# Autodesk Inventor assembly: Mechanizm
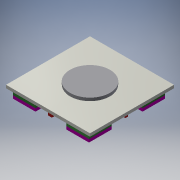
[picture p0: Inventor's stored thumbnail of the model, 180x180]
Saved by Autodesk Inventor 2018 (Build 220112000, 112)
## iProperties
Created: 2018-10-22
Part Number: Mechanizm
Material: Ogólny
Document SubType Name: Assembly
Designer: EWA
Author: EWA
## Documents named in this file (7)
- C:\Users\EWA\Documents\Inventor\Kostka\Mechanizm.iam
- C:\Users\EWA\Documents\Inventor\Kostka\Zamek_II_klucz.ipt
- C:\Users\EWA\Documents\Inventor\Kostka\Pokrywka.ipt
- C:\Users\EWA\Documents\Inventor\Kostka\zamek_II_boki.ipt
- C:\Users\EWA\Documents\Inventor\Kostka\Zamek_I.ipt
- C:\Users\EWA\Documents\Inventor\Kostka\Sciana_pokrywka_168x168.ipt
- C:\Users\EWA\Documents\Inventor\Kostka\Uchwyt_80.ipt
## Components (9 placed, 6 different names)
1. Pokrywka:1 — Zestawiający:1, Równoległy:1, Równoległy:2, Obrotowe:1, Zestawiający:2, Zestawiający:3, Równoległy:3, Równoległy:4, Równoległy:5, Równoległy:6, Zestawiający:4, Zestawiający:5, Równoległy:7, Równoległy:8
2. Zamek_II_klucz:1 — Obrotowe:1
3. zamek_II_boki:1 — Zestawiający:3, Równoległy:3, Równoległy:4
4. zamek_II_boki:2 — Równoległy:1, Równoległy:2, Zestawiający:4, Równoległy:10
5. zamek_II_boki:3 — Zestawiający:2, Równoległy:5, Równoległy:6, Zestawiający:6
6. zamek_II_boki:4 — Zestawiający:1, Zestawiający:5, Równoległy:7, Równoległy:8, Równoległy:9
7. Zamek_I:1 — Zestawiający:6, Równoległy:9, Równoległy:10, Równoległy:11, Równoległy:12, Zestawiający:7
8. Sciana_pokrywka_168x168:1 — Równoległy:11, Równoległy:12, Obrotowe:2, Zestawiający:7
9. Uchwyt_80:1 — Obrotowe:2
## Relationships (21: Flush 12, Mate 7, RevoluteJoint 2)
- Zestawiający:1 [Mate]: Pokrywka:1 ↔ zamek_II_boki:4
- Równoległy:1 [Flush]: Pokrywka:1 ↔ zamek_II_boki:2
- Równoległy:2 [Flush]: Pokrywka:1 ↔ zamek_II_boki:2
- Obrotowe:1 [RevoluteJoint]: Pokrywka:1 ↔ Zamek_II_klucz:1
- Zestawiający:2 [Mate]: Pokrywka:1 ↔ zamek_II_boki:3
- Zestawiający:3 [Mate]: Pokrywka:1 ↔ zamek_II_boki:1
- Równoległy:3 [Flush]: Pokrywka:1 ↔ zamek_II_boki:1
- Równoległy:4 [Flush]: Pokrywka:1 ↔ zamek_II_boki:1
- Równoległy:5 [Flush]: Pokrywka:1 ↔ zamek_II_boki:3
- Równoległy:6 [Flush]: Pokrywka:1 ↔ zamek_II_boki:3
- Zestawiający:4 [Mate]: Pokrywka:1 ↔ zamek_II_boki:2
- Zestawiający:5 [Mate]: Pokrywka:1 ↔ zamek_II_boki:4
- Równoległy:7 [Flush]: Pokrywka:1 ↔ zamek_II_boki:4
- Równoległy:8 [Flush]: Pokrywka:1 ↔ zamek_II_boki:4
- Zestawiający:6 [Mate]: zamek_II_boki:3 ↔ Zamek_I:1
- Równoległy:9 [Flush]: zamek_II_boki:4 ↔ Zamek_I:1
- Równoległy:10 [Flush]: zamek_II_boki:2 ↔ Zamek_I:1
- Równoległy:11 [Flush] (-9 mm): Zamek_I:1 ↔ Sciana_pokrywka_168x168:1
- Równoległy:12 [Flush] (-9 mm): Zamek_I:1 ↔ Sciana_pokrywka_168x168:1
- Obrotowe:2 [RevoluteJoint]: Sciana_pokrywka_168x168:1 ↔ Uchwyt_80:1
- Zestawiający:7 [Mate]: Zamek_I:1 ↔ Sciana_pokrywka_168x168:1
